# Autodesk Inventor assembly: HS 60T Gear, Circle Insert
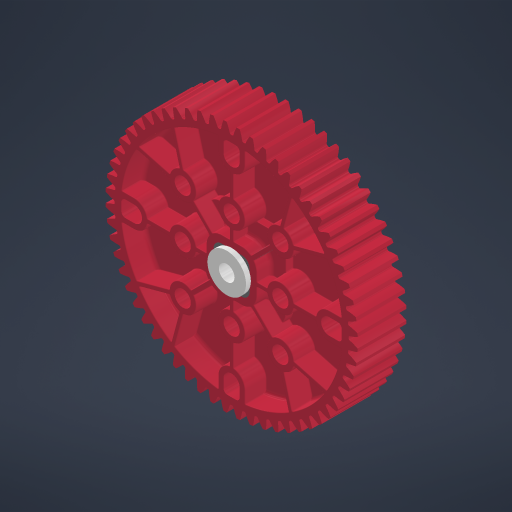
[picture p0: Inventor's stored thumbnail of the model, 512x512]
Saved by Autodesk Inventor 2024 (Build 280153000, 153)
## iProperties
Created: 2023-08-12
Part Number: HS 60T Gear, Circle Insert
Document SubType Name: Assembly
Designer: macbook
Author: macbook
## Documents named in this file (4)
- \\Mac\Home\Desktop\code\7899V-VRC-OVER-UNDER\Cad\VEX-CAD-Inventor-1.4.0\Motion\Gears\HS Gear\HS 60T Gear, Circle Insert.iam
- \\Mac\Home\Desktop\code\7899V-VRC-OVER-UNDER\Cad\VEX-CAD-Inventor-1.4.0\Motion\Gears\HS Gear.iam
- \\Mac\Home\Desktop\code\7899V-VRC-OVER-UNDER\Cad\VEX-CAD-Inventor-1.4.0\Motion\Gears\HS Gear\HS 60T Gear, No Insert.iam
- \\Mac\Home\Desktop\code\7899V-VRC-OVER-UNDER\Cad\VEX-CAD-Inventor-1.4.0\Motion\Insert Circle.ipt
## Components (3 placed, 2 different names)
1. HS 60T Gear, No Insert:1 [sub-assembly] — Insert:1, Insert:2
2. Insert Circle:1 — Insert:1
3. Insert Circle:2 — Insert:2
## Relationships (2: Insert 2)
- Insert:1: HS 60T Gear, No Insert:1 ↔ Insert Circle:1
- Insert:2: HS 60T Gear, No Insert:1 ↔ Insert Circle:2
